# Autodesk Inventor assembly: RailAndMirror
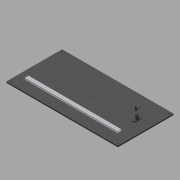
[picture p0: Inventor's stored thumbnail of the model, 180x180]
Saved by Autodesk Inventor 2018 (Build 220112000, 112)
## iProperties
Created: 2018-09-17
Part Number: RailAndMirror
Document SubType Name: Assembly
Designer: Robert Campbell
Author: Robert Campbell
## Documents named in this file (4)
- X:\home\work\Documents\MF_BenchOptics\CAD_files\RailAndMirror.iam
- X:\home\work\Documents\MF_BenchOptics\CAD_files\MB60120_M-Solidworks.ipt
- X:\home\work\Documents\MF_BenchOptics\CAD_files\XT66DP-1000-Solidworks.ipt
- X:\home\work\Documents\MF_BenchOptics\CAD_files\first_mirror.iam
## Components (3 placed, 3 different names)
1. MB60120_M-Solidworks:1 — Mate:1, Mate:21, Angle:4
2. XT66DP-1000-Solidworks:1 — Mate:1
3. first_mirror:1 [sub-assembly] — Mate:21, Angle:4
## Relationships (3: Mate 2, Angle 1)
- Mate:1: MB60120_M-Solidworks:1 ↔ XT66DP-1000-Solidworks:1
- Mate:21: MB60120_M-Solidworks:1 ↔ first_mirror:1
- Angle:4 (0 deg): MB60120_M-Solidworks:1 ↔ first_mirror:1
